# Autodesk Inventor assembly: REAL_Upright_Assembly_V1
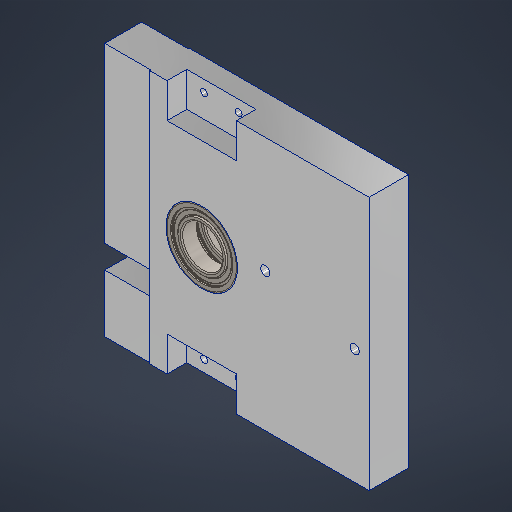
[picture p0: Inventor's stored thumbnail of the model, 512x512]
Saved by Autodesk Inventor 2026.1 (Build 301233000, 233)
## iProperties
Created: 2026-09-05
Part Number: REAL_Upright_Assembly_V1
Document SubType Name: Assembly
Designer: share
Author: share
## Documents named in this file (3)
- C:\Users\share\OneDrive\Documents\Personal Projects\GOGO Kart\CAD\GOGO_KART_FSAE\Suspension\REAL Upright\REAL_Upright_Assembly_V1.iam
- C:\Users\share\OneDrive\Documents\Personal Projects\GOGO Kart\CAD\GOGO_KART_FSAE\Suspension\REAL Upright\Suspension_Upright_V2_Topology Baseline.ipt
- C:\Users\share\Downloads\grainger-35hz68\grainger-35hz68\grainger-35hz68\grainger-35hz68.ipt
## Components (3 placed, 2 different names)
1. Suspension_Upright_V2_Topology Baseline:1 — Flush:1, Flush:2, Flush:3, Insert:1, Insert:2
2. grainger-35hz68:1 — Insert:1
3. grainger-35hz68:2 — Insert:2
## Relationships (5: Flush 3, Insert 2)
- Flush:1: Suspension_Upright_V2_Topology Baseline:1
- Flush:2: Suspension_Upright_V2_Topology Baseline:1
- Flush:3: Suspension_Upright_V2_Topology Baseline:1
- Insert:1: Suspension_Upright_V2_Topology Baseline:1 ↔ grainger-35hz68:1
- Insert:2: Suspension_Upright_V2_Topology Baseline:1 ↔ grainger-35hz68:2
